# Autodesk Inventor assembly: W13-3
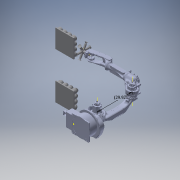
[picture p0: Inventor's stored thumbnail of the model, 180x180]
Saved by Autodesk Inventor 2017 (Build 210142000, 142)
## iProperties
Created: 2020-12-29
Part Number: W13-3
Material: 一般
Document SubType Name: Assembly
Designer: Brian
Sending System: Autodesk Inventor 2020
Preprocessor: ST-DEVELOPER v18
Title: F:\DesktopSpace\MASTERS\ma2010_asm.stp
Author: Crowm
Revision Number: ANY
## Documents named in this file (11)
- E:\coppeliaSim\3D\機械手臂 3D\W13-3.iam
- E:\coppeliaSim\3D\機械手臂 3D\BASE_AXIS.ipt
- E:\coppeliaSim\3D\機械手臂 3D\S_AXIS.ipt
- E:\coppeliaSim\3D\機械手臂 3D\L_AXIS.ipt
- E:\coppeliaSim\3D\機械手臂 3D\U_AXIS.ipt
- E:\coppeliaSim\3D\機械手臂 3D\R_AXIS.ipt
- E:\coppeliaSim\3D\機械手臂 3D\B_AXIS.ipt
- E:\coppeliaSim\3D\機械手臂 3D\T_AXIS.ipt
- E:\coppeliaSim\3D\機械手臂 3D\六針夾爪.ipt
- E:\coppeliaSim\3D\機械手臂 3D\球底座.ipt
- E:\coppeliaSim\3D\機械手臂 3D\球.ipt
## Components (40 placed, 10 different names)
1. BASE_AXIS_433 — 貼合:1, 貼合:2, Angle:1
2. S_AXIS_434 — 貼合:1, 貼合:2, 貼合:3, 貼合:4, Angle:3
3. L_AXIS_435 — 貼合:3, 貼合:4, 貼合:5, 貼合:6, Angle:1, Angle:2
4. U_AXIS_436 — 貼合:5, 貼合:6, 貼合:7, 貼合:8, Angle:2, Angle:3, Angle:4
5. R_AXIS_437 — 貼合:7, 貼合:8, 貼合:9, Mate:14, Angle:4, Angle:5, Angle:6
6. B_AXIS_438 — 貼合:9, 貼合:11, 貼合:12, Mate:14, Flush:1, Angle:5
7. T_AXIS_439 — 貼合:11, 貼合:12, Mate:15
8. 六針夾爪:1 — Mate:15, Flush:1, Angle:6
9. 球底座:1 — Mate:16, Mate:17, Mate:18, Mate:19, Mate:20, Mate:21, Mate:22, Mate:23, Mate:24, Mate:25, Mate:26, Mate:27, Mate:28, Mate:29, Mate:30, Mate:31, Flush:3, Flush:4, Mate:33
10. 球:1 — Mate:20, Tangent:5, Tangent:7
11. 球:2 — Mate:18, Tangent:3, Tangent:11
12. 球:3 — Mate:17, Tangent:2, Tangent:4
13. 球:4 — Mate:16, Tangent:1
14. 球:5 — Mate:19, Tangent:10
15. 球:6 — Tangent:1, Tangent:2, Tangent:3, Tangent:19
16. 球:7 — Mate:21, Tangent:6, Tangent:13, Tangent:16
17. 球:8 — Mate:24, Tangent:12, Tangent:25
18. 球:9 — Tangent:7, Tangent:8, Tangent:9, Tangent:24
19. 球:10 — Mate:23, Tangent:8, Tangent:18
20. 球:11 — Mate:22, Tangent:9
21. 球:12 — Tangent:4, Tangent:5, Tangent:6, Tangent:21, Tangent:22
22. 球:13 — Mate:25, Tangent:15, Tangent:26, Tangent:34
23. 球:14 — Mate:27, Tangent:36
24. 球:15 — Mate:28, Tangent:14, Tangent:17, Tangent:33, Tangent:35
25. 球:16 — Mate:26, Tangent:27
26. 球:17 — Tangent:28, Tangent:29, Tangent:30
27. 球:18 — Tangent:37, Tangent:38, Tangent:39, Tangent:41
28. 球:19 — Mate:31, Tangent:31
29. 球:20 — Tangent:25, Tangent:26, Tangent:27, Tangent:28
30. 球:22 — Tangent:31, Tangent:32, Tangent:33, Tangent:39
31. 球:23 — Tangent:40, Tangent:41, Tangent:42
32. 球:25 — Tangent:34, Tangent:35, Tangent:36
33. 球:27 — Tangent:22, Tangent:23, Tangent:24, Tangent:42
34. 球:28 — Tangent:13, Tangent:14, Tangent:15, Tangent:23, Tangent:30, Tangent:37
35. 球:29 — Tangent:16, Tangent:17, Tangent:18, Tangent:38
36. 球:30 — Tangent:19, Tangent:20, Tangent:21, Tangent:40
37. 球:31 — Tangent:10, Tangent:11, Tangent:12, Tangent:20, Tangent:29
38. 球:32 — Mate:30, Tangent:32
39. 球:33 — Mate:29
40. 球底座:2 — Flush:3, Flush:4, Mate:33
## Relationships (81: Tangent 42, Mate 30, Angle 6, Flush 3)
- 貼合:1 [Mate]: BASE_AXIS_433 ↔ S_AXIS_434
- 貼合:2 [Mate]: BASE_AXIS_433 ↔ S_AXIS_434
- 貼合:3 [Mate]: S_AXIS_434 ↔ L_AXIS_435
- 貼合:4 [Mate]: S_AXIS_434 ↔ L_AXIS_435
- 貼合:5 [Mate]: L_AXIS_435 ↔ U_AXIS_436
- 貼合:6 [Mate]: L_AXIS_435 ↔ U_AXIS_436
- 貼合:7 [Mate]: U_AXIS_436 ↔ R_AXIS_437
- 貼合:8 [Mate]: U_AXIS_436 ↔ R_AXIS_437
- 貼合:9 [Mate]: R_AXIS_437 ↔ B_AXIS_438
- 貼合:11 [Mate]: B_AXIS_438 ↔ T_AXIS_439
- 貼合:12 [Mate]: B_AXIS_438 ↔ T_AXIS_439
- Mate:14: R_AXIS_437 ↔ B_AXIS_438
- Mate:15: T_AXIS_439 ↔ 六針夾爪:1
- Flush:1: B_AXIS_438 ↔ 六針夾爪:1
- Mate:16: 球底座:1 ↔ 球:4
- Mate:17: 球底座:1 ↔ 球:3
- Mate:18: 球底座:1 ↔ 球:2
- Mate:19: 球底座:1 ↔ 球:5
- Tangent:1: 球:4 ↔ 球:6
- Tangent:2: 球:3 ↔ 球:6
- Tangent:3: 球:2 ↔ 球:6
- Mate:20: 球底座:1 ↔ 球:1
- Mate:21: 球底座:1 ↔ 球:7
- Mate:22: 球底座:1 ↔ 球:11
- Mate:23: 球底座:1 ↔ 球:10
- Tangent:4: 球:3 ↔ 球:12
- Tangent:5: 球:1 ↔ 球:12
- Tangent:6: 球:7 ↔ 球:12
- Tangent:7: 球:1 ↔ 球:9
- Tangent:8: 球:9 ↔ 球:10
- Tangent:9: 球:9 ↔ 球:11
- Mate:24: 球底座:1 ↔ 球:8
- Mate:25: 球底座:1 ↔ 球:13
- Mate:26: 球底座:1 ↔ 球:16
- Mate:27: 球底座:1 ↔ 球:14
- Mate:28: 球底座:1 ↔ 球:15
- Mate:29: 球底座:1 ↔ 球:33
- Mate:30: 球底座:1 ↔ 球:32
- Mate:31: 球底座:1 ↔ 球:19
- Tangent:10: 球:5 ↔ 球:31
- Tangent:11: 球:2 ↔ 球:31
- Tangent:12: 球:8 ↔ 球:31
- Tangent:13: 球:7 ↔ 球:28
- Tangent:14: 球:15 ↔ 球:28
- Tangent:15: 球:13 ↔ 球:28
- Tangent:16: 球:7 ↔ 球:29
- Tangent:17: 球:15 ↔ 球:29
- Tangent:18: 球:10 ↔ 球:29
- Tangent:19: 球:6 ↔ 球:30
- Tangent:20: 球:30 ↔ 球:31
- Tangent:21: 球:12 ↔ 球:30
- Tangent:22: 球:12 ↔ 球:27
- Tangent:23: 球:27 ↔ 球:28
- Tangent:24: 球:9 ↔ 球:27
- Tangent:25: 球:8 ↔ 球:20
- Tangent:26: 球:13 ↔ 球:20
- Tangent:27: 球:16 ↔ 球:20
- Tangent:28: 球:17 ↔ 球:20
- Tangent:29: 球:17 ↔ 球:31
- Tangent:30: 球:17 ↔ 球:28
- Tangent:31: 球:19 ↔ 球:22
- Tangent:32: 球:22 ↔ 球:32
- Tangent:33: 球:15 ↔ 球:22
- Tangent:34: 球:13 ↔ 球:25
- Tangent:35: 球:15 ↔ 球:25
- Tangent:36: 球:14 ↔ 球:25
- Tangent:37: 球:18 ↔ 球:28
- Tangent:38: 球:18 ↔ 球:29
- Tangent:39: 球:18 ↔ 球:22
- Tangent:40: 球:23 ↔ 球:30
- Tangent:41: 球:18 ↔ 球:23
- Tangent:42: 球:23 ↔ 球:27
- Flush:3: 球底座:1 ↔ 球底座:2
- Flush:4: 球底座:1 ↔ 球底座:2
- Mate:33 (600 mm): 球底座:1 ↔ 球底座:2
- Angle:1 (180 deg): BASE_AXIS_433 ↔ L_AXIS_435
- Angle:2 (0 deg): L_AXIS_435 ↔ U_AXIS_436
- Angle:3 (0 deg): S_AXIS_434 ↔ U_AXIS_436
- Angle:4 (0 deg): U_AXIS_436 ↔ R_AXIS_437
- Angle:5 (0 deg): R_AXIS_437 ↔ B_AXIS_438
- Angle:6 (0 deg): R_AXIS_437 ↔ 六針夾爪:1
